# Autodesk Inventor assembly: CarAssembly
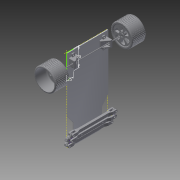
[picture p0: Inventor's stored thumbnail of the model, 180x180]
Saved by Autodesk Inventor 2015 (Build 190159000, 159)
## iProperties
Created: 2014-11-05
Part Number: CarAssembly
Document SubType Name: Assembly
Designer: ah14592
Author: ah14592
## Documents named in this file (9)
- C:\Users\ah14592\Desktop\Inventor\Assembly\CarAssembly.iam
- C:\Users\ah14592\Desktop\Inventor\Rear Axel Holder\holder1.ipt
- C:\Users\ah14592\Desktop\Inventor\RearAxel.ipt
- C:\Users\ah14592\Desktop\Inventor\Base\Basetrimed.ipt
- C:\Users\ah14592\Desktop\Inventor\Rear Axel Holder\holder1_MIR1.ipt
- C:\Users\ah14592\Desktop\Inventor\Wheels\Rear Wheels\Wheels1.ipt
- C:\Users\ah14592\Desktop\Inventor\Steering\Steering Rod\mk1.ipt
- C:\Users\ah14592\Desktop\Inventor\Steering\Steering T\Part3.ipt
- C:\Users\ah14592\Desktop\Inventor\Steering\T Connector Rod\Part1.ipt
## Components (11 placed, 8 different names)
1. holder 1 — Mate:3, Flush:1, Flush:2, Mate:4, Flush:5
2. Basetrimed:1 — Mate:3, Flush:1, Flush:2, Flush:3, Flush:4, Flush:8, Mate:7, Flush:9
3. holder1_MIR1:1 — Flush:3, Flush:4
4. Wheels1:1 — Mate:6, Flush:6
5. Wheels1:2 — Mate:5, Flush:7
6. RearAxel:1 — Mate:4, Mate:5, Mate:6, Flush:5, Flush:6, Flush:7
7. mk1:1 — Mate:14, Mate:15, Mate:16
8. mk1:2 — Mate:12, Mate:13, Mate:17
9. Part3:1 — Mate:8, Mate:9, Mate:12, Mate:13, Mate:14, Mate:15
10. Part3:2 — Mate:10, Mate:11, Mate:16, Mate:17
11. Part1:1 — Flush:8, Mate:7, Flush:9, Mate:8, Mate:9, Mate:10, Mate:11
## Relationships (24: Mate 15, Flush 9)
- Mate:3: holder 1 ↔ Basetrimed:1
- Flush:1 (5 mm): holder 1 ↔ Basetrimed:1
- Flush:2 (8 mm): holder 1 ↔ Basetrimed:1
- Flush:3 (5 mm): Basetrimed:1 ↔ holder1_MIR1:1
- Flush:4 (8 mm): Basetrimed:1 ↔ holder1_MIR1:1
- Mate:4: holder 1 ↔ RearAxel:1
- Mate:5: Wheels1:2 ↔ RearAxel:1
- Mate:6: Wheels1:1 ↔ RearAxel:1
- Flush:5 (56 mm): holder 1 ↔ RearAxel:1
- Flush:6 (-8 mm): Wheels1:1 ↔ RearAxel:1
- Flush:7 (-8 mm): Wheels1:2 ↔ RearAxel:1
- Flush:8 (-25 mm): Basetrimed:1 ↔ Part1:1
- Mate:7: Basetrimed:1 ↔ Part1:1
- Flush:9 (-34.5 mm): Basetrimed:1 ↔ Part1:1
- Mate:8: Part3:1 ↔ Part1:1
- Mate:9: Part3:1 ↔ Part1:1
- Mate:10: Part3:2 ↔ Part1:1
- Mate:11: Part3:2 ↔ Part1:1
- Mate:12: mk1:2 ↔ Part3:1
- Mate:13: mk1:2 ↔ Part3:1
- Mate:14: mk1:1 ↔ Part3:1
- Mate:15: mk1:1 ↔ Part3:1
- Mate:16: mk1:1 ↔ Part3:2
- Mate:17: mk1:2 ↔ Part3:2
